# Autodesk Inventor assembly: TankFlipperAssembledDriveShaft
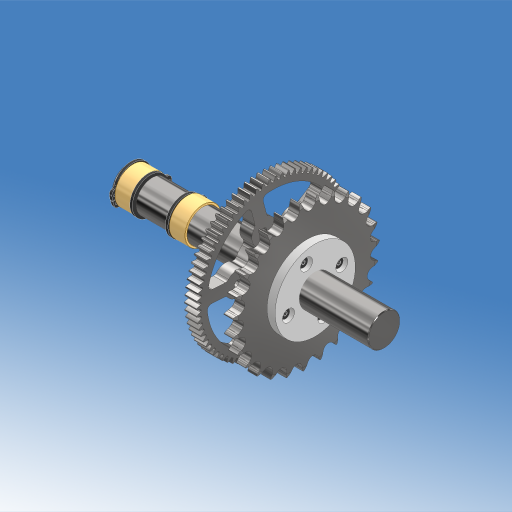
[picture p0: Inventor's stored thumbnail of the model, 512x512]
Saved by Autodesk Inventor 2024 (Build 280153000, 153)
## iProperties
Created: 2024-02-13
Part Number: TankFlipperAssembledDriveShaft
Document SubType Name: Assembly
Designer: seene
Author: seene
## Documents named in this file (9)
- C:\Users\seene\OneDrive\SBRT\Robocup Rescue\Drive\v1\TANK flipper\TankFlipperAssembledDriveShaft - newTrack.iam
- C:\Users\seene\OneDrive\SBRT\Robocup Rescue\Drive\v1\TANK flipper\Drive Shaft.ipt
- C:\Users\seene\OneDrive\SBRT\Robocup Rescue\Drive\v1\TANK flipper\98585A121_Heavy Duty External Retaining Ring v2.ipt
- C:\Users\seene\OneDrive\SBRT\Robocup Rescue\Drive\v1\TANK flipper\2868T199_High-Load Oil-Embedded 863 Sleeve Bearing (1) v2(Mirror).ipt
- C:\Users\seene\OneDrive\SBRT\Robocup Rescue\Drive\v1\TANK flipper\27t track drive sprocket v25.iam
- C:\Users\seene\OneDrive\SBRT\Robocup Rescue\Drive\v1\TANK flipper\Spur Gear (74 teeth).ipt
- C:\Users\seene\OneDrive\SBRT\Robocup Rescue\Drive\v1\TANK flipper\panel_flange.ipt
- C:\Users\seene\OneDrive\SBRT\Robocup Rescue\Drive\v1\TANK flipper\bushing_2868T199.ipt
- C:\Users\seene\OneDrive\SBRT\Robocup Rescue\Drive\v1\TANK flipper\94328A911_Black Oxide Alloy Steel Low-Profile Shoulder Screw v2.ipt
## Components (18 placed, 8 different names)
1. Drive Shaft:1 — Rigid:1, Rigid:2, Rigid:3, Rigid:4, Rigid:5, Rigid:17, Mate:6
2. 98585A121_Heavy Duty External Retaining Ring v2:1 — Rigid:1
3. 2868T199_High-Load Oil-Embedded 863 Sleeve Bearing (1) v2(Mirror):1 — Rigid:2, Rigid:18
4. 27t track drive sprocket v25:1 [sub-assembly] — Rigid:4
5. 98585A121_Heavy Duty External Retaining Ring v2:2 — Rigid:3
6. 98585A121_Heavy Duty External Retaining Ring v2:3 — Rigid:5
7. Spur Gear (74 teeth):1 — Rigid:16
8. panel_flange:1 — Rigid:18
9. panel_flange:2 — Mate:3, Mate:4, Mate:5, Rigid:25
10. bushing_2868T199:1 — Rigid:16, Rigid:26, Mate:6
11. bushing_2868T199:2 — Rigid:26, Rotational:1
12. bushing_2868T199:3 — Rigid:17, Rigid:25
13. 27t track drive sprocket v25:2 [sub-assembly] — Rotational:1
14. 94328A911_Black Oxide Alloy Steel Low-Profile Shoulder Screw v2:1 — Mate:5
15. 94328A911_Black Oxide Alloy Steel Low-Profile Shoulder Screw v2:2
16. 94328A911_Black Oxide Alloy Steel Low-Profile Shoulder Screw v2:3
17. 94328A911_Black Oxide Alloy Steel Low-Profile Shoulder Screw v2:4 — Mate:3, Mate:4
18. 94328A911_Black Oxide Alloy Steel Low-Profile Shoulder Screw v2:5
## Relationships (15: WeldJoint 10, Mate 4, RevoluteJoint 1)
- Rigid:1 [WeldJoint]: Drive Shaft:1 ↔ 98585A121_Heavy Duty External Retaining Ring v2:1
- Rigid:2 [WeldJoint]: Drive Shaft:1 ↔ 2868T199_High-Load Oil-Embedded 863 Sleeve Bearing (1) v2(Mirror):1
- Rigid:3 [WeldJoint]: Drive Shaft:1 ↔ 98585A121_Heavy Duty External Retaining Ring v2:2
- Rigid:4 [WeldJoint]: Drive Shaft:1 ↔ 27t track drive sprocket v25:1
- Rigid:5 [WeldJoint]: Drive Shaft:1 ↔ 98585A121_Heavy Duty External Retaining Ring v2:3
- Rigid:16 [WeldJoint]: Spur Gear (74 teeth):1 ↔ bushing_2868T199:1
- Rigid:17 [WeldJoint]: Drive Shaft:1 ↔ bushing_2868T199:3
- Rigid:18 [WeldJoint]: 2868T199_High-Load Oil-Embedded 863 Sleeve Bearing (1) v2(Mirror):1 ↔ panel_flange:1
- Mate:3: panel_flange:2 ↔ 94328A911_Black Oxide Alloy Steel Low-Profile Shoulder Screw v2:4
- Mate:4: panel_flange:2 ↔ 94328A911_Black Oxide Alloy Steel Low-Profile Shoulder Screw v2:4
- Mate:5: panel_flange:2 ↔ 94328A911_Black Oxide Alloy Steel Low-Profile Shoulder Screw v2:1
- Rigid:25 [WeldJoint]: panel_flange:2 ↔ bushing_2868T199:3
- Rigid:26 [WeldJoint]: bushing_2868T199:1 ↔ bushing_2868T199:2
- Rotational:1 [RevoluteJoint]: bushing_2868T199:2 ↔ 27t track drive sprocket v25:2
- Mate:6: Drive Shaft:1 ↔ bushing_2868T199:1
